# Autodesk Inventor assembly: beepanda
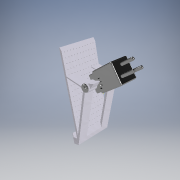
[picture p0: Inventor's stored thumbnail of the model, 180x180]
Saved by Autodesk Inventor 2019 (Build 230136000, 136)
## iProperties
Created: 2020-04-08
Part Number: beepanda
Document SubType Name: Assembly
Designer: Manoj
Author: Manoj
## Documents named in this file (4)
- F:\Softwares\Autodesk\Inventor projects\beepanda.iam
- F:\Softwares\Autodesk\Inventor projects\bee pindi.ipt
- F:\Softwares\Autodesk\Inventor projects\bee poo.ipt
- F:\Softwares\Autodesk\Inventor projects\panda.ipt
## Components (3 placed, 3 different names)
1. bee pindi:1 — Mate:1, Mate:2, Cylindrical:1, Cylindrical:2, Mate:3, Mate:4, Mate:5
2. bee poo:1 — Mate:1, Mate:2, Cylindrical:1, Cylindrical:2, Mate:3
3. panda:1 — Mate:4, Mate:5
## Relationships (7: Mate 5, CylindricalJoint 2)
- Mate:1 (3.81 mm): bee pindi:1 ↔ bee poo:1
- Mate:2: bee pindi:1 ↔ bee poo:1
- Cylindrical:1: bee pindi:1 ↔ bee poo:1
- Cylindrical:2: bee pindi:1 ↔ bee poo:1
- Mate:3: bee pindi:1 ↔ bee poo:1
- Mate:4: bee pindi:1 ↔ panda:1
- Mate:5: bee pindi:1 ↔ panda:1
